# Autodesk Inventor assembly: Shoulder
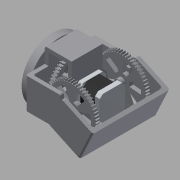
[picture p0: Inventor's stored thumbnail of the model, 180x180]
Saved by Autodesk Inventor 2017 (Build 210142000, 142)
## iProperties
Created: 2017-05-07
Part Number: Shoulder
Document SubType Name: Assembly
Designer: zallen
Author: zallen
## Documents named in this file (10)
- C:\Users\zallen\Documents\Autodesk Inventor Projects\LaundryRobot_v0.1\Arm\Shoulder\Shoulder.iam
- C:\Users\zallen\Documents\Autodesk Inventor Projects\LaundryRobot_v0.1\Arm\Shoulder\ShoulderGearYZ.ipt
- C:\Users\zallen\Documents\Autodesk Inventor Projects\LaundryRobot_v0.1\Arm\Shoulder\ShoulderPlateXZ.ipt
- C:\Users\zallen\Documents\Autodesk Inventor Projects\Stepper Motor\Двигатель.ipt
- C:\Users\zallen\Documents\Autodesk Inventor Projects\LaundryRobot_v0.1\Arm\Shoulder\Gear.ipt
- C:\Users\zallen\Documents\Autodesk Inventor Projects\LaundryRobot_v0.1\Arm\Shoulder\Shoulder\Design Accelerator\Bolted Connection3.iam
- C:\Users\zallen\Documents\Autodesk Inventor Projects\LaundryRobot_v0.1\Arm\Shoulder\Shoulder\Design Accelerator\Bolted Connection4.iam
- C:\Users\zallen\Documents\Autodesk Inventor Projects\LaundryRobot_v0.1\Arm\Shoulder\Shoulder\Design Accelerator\Bolted Connection5.iam
- C:\Users\zallen\Documents\Autodesk Inventor Projects\LaundryRobot_v0.1\Arm\Shoulder\Shoulder\Design Accelerator\Bolted Connection6.iam
- C:\Users\zallen\Documents\Autodesk Inventor Projects\LaundryRobot_v0.1\Arm\Shoulder\Bracket3.ipt
## Components (11 placed, 6 different names)
1. ShoulderGearYZ:1 — Flush:1, Mate:3, Mate:4, Mate:8, Mate:12
2. ShoulderPlateXZ:1 — Flush:1, Mate:1, Mate:2, Mate:3, Mate:4, Mate:5, Mate:6, Mate:7, Mate:9, Mate:10, Mate:11, Mate:19, Mate:20, Mate:21
3. StepperMotor:1 — Mate:13, Mate:14
4. Gear:1 — Mate:1, Mate:2, Mate:13, Mate:14
5. Bolted Connection:1 [sub-assembly] — Mate:5, Mate:6
6. Bolted Connection:2 [sub-assembly] — Mate:7, Mate:8
7. Bolted Connection:3 [sub-assembly] — Mate:9, Mate:10
8. Bolted Connection:4 [sub-assembly] — Mate:11, Mate:12
9. Gear:2 — Mate:15, Mate:16
10. Bracket3:1 — Mate:15, Mate:16, Mate:17, Mate:18, Mate:20, Mate:21
11. Gear:3 — Mate:17, Mate:18, Mate:19
## Relationships (22: Mate 21, Flush 1)
- Flush:1: ShoulderGearYZ:1 ↔ ShoulderPlateXZ:1
- Mate:1: ShoulderPlateXZ:1 ↔ Gear:1
- Mate:2: ShoulderPlateXZ:1 ↔ Gear:1
- Mate:3: ShoulderGearYZ:1 ↔ ShoulderPlateXZ:1
- Mate:4: ShoulderGearYZ:1 ↔ ShoulderPlateXZ:1
- Mate:5: ShoulderPlateXZ:1 ↔ Bolted Connection:1
- Mate:6: ShoulderPlateXZ:1 ↔ Bolted Connection:1
- Mate:7: ShoulderPlateXZ:1 ↔ Bolted Connection:2
- Mate:8: ShoulderGearYZ:1 ↔ Bolted Connection:2
- Mate:9: ShoulderPlateXZ:1 ↔ Bolted Connection:3
- Mate:10: ShoulderPlateXZ:1 ↔ Bolted Connection:3
- Mate:11: ShoulderPlateXZ:1 ↔ Bolted Connection:4
- Mate:12: ShoulderGearYZ:1 ↔ Bolted Connection:4
- Mate:13: StepperMotor:1 ↔ Gear:1
- Mate:14: StepperMotor:1 ↔ Gear:1
- Mate:15: Gear:2 ↔ Bracket3:1
- Mate:16: Gear:2 ↔ Bracket3:1
- Mate:17: Bracket3:1 ↔ Gear:3
- Mate:18: Bracket3:1 ↔ Gear:3
- Mate:19: ShoulderPlateXZ:1 ↔ Gear:3
- Mate:20: ShoulderPlateXZ:1 ↔ Bracket3:1
- Mate:21: ShoulderPlateXZ:1 ↔ Bracket3:1
